# Autodesk Inventor assembly: FrameV4
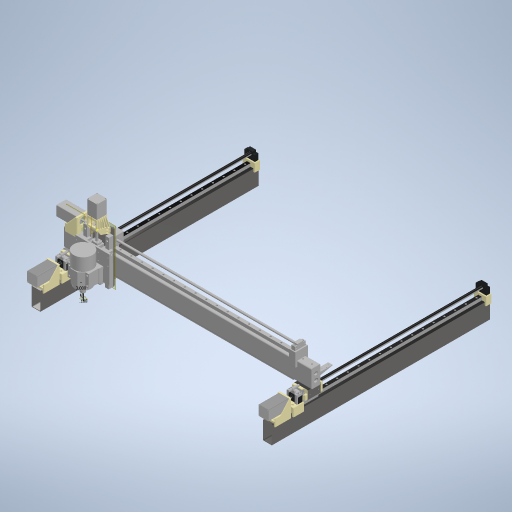
[picture p0: Inventor's stored thumbnail of the model, 512x512]
Saved by Autodesk Inventor 2023 (Build 270158000, 158)
## iProperties
Created: 2022-05-07
Part Number: FrameV4
Document SubType Name: Assembly
Designer: plebbb
Mass: 10930.1 g
Surface Area: 33660.3 cm^2
Volume: 10930.1 cm^3
Density: 1 g/cm^3
Author: plebbb
## Documents named in this file (4)
- D:\Users\plebbb\Desktop\CNC_Project\FrameV4.iam
- D:\Users\plebbb\Desktop\CNC_Project\Ballscrew_Assembly.iam
- D:\Users\plebbb\Desktop\CNC_Project\X_GANTRY.iam
- D:\Users\plebbb\Desktop\CNC_Project\YZ_GANTRY.iam
## Components (5 placed, 3 different names)
1. Ballscrew_Assembly:1 [sub-assembly] — Mate:84
2. Ballscrew_Assembly:2 [sub-assembly] — Mate:83, Mate:85, Mate:86
3. X_GANTRY:1 [sub-assembly] — Mate:80, Mate:81, Mate:82, Flush:21, Flush:22, Mate:83, Mate:85, Mate:86
4. X_GANTRY:2 [sub-assembly] — Flush:21, Flush:22, Mate:84
5. YZ_GANTRY:1 [sub-assembly]
## Relationships (15: Mate 13, Flush 2)
- [Mate]: Ballscrew_Assembly:1 ↔ YZ_GANTRY:1
- [Mate]: Ballscrew_Assembly:1 ↔ YZ_GANTRY:1
- [Mate]: Ballscrew_Assembly:2 ↔ YZ_GANTRY:1
- [Mate]: Ballscrew_Assembly:2 ↔ YZ_GANTRY:1
- [Mate]: Ballscrew_Assembly:1 ↔ YZ_GANTRY:1
- [Mate]: Ballscrew_Assembly:2 ↔ YZ_GANTRY:1
- Mate:80: X_GANTRY:1
- Mate:81: X_GANTRY:1
- Mate:82: X_GANTRY:1
- Flush:21: X_GANTRY:1 ↔ X_GANTRY:2
- Flush:22: X_GANTRY:1 ↔ X_GANTRY:2
- Mate:83: Ballscrew_Assembly:2 ↔ X_GANTRY:1
- Mate:84: Ballscrew_Assembly:1 ↔ X_GANTRY:2
- Mate:85: Ballscrew_Assembly:2 ↔ X_GANTRY:1
- Mate:86: Ballscrew_Assembly:2 ↔ X_GANTRY:1
